# Autodesk Inventor assembly: STI Hybrid 98 Full Flange Assembly
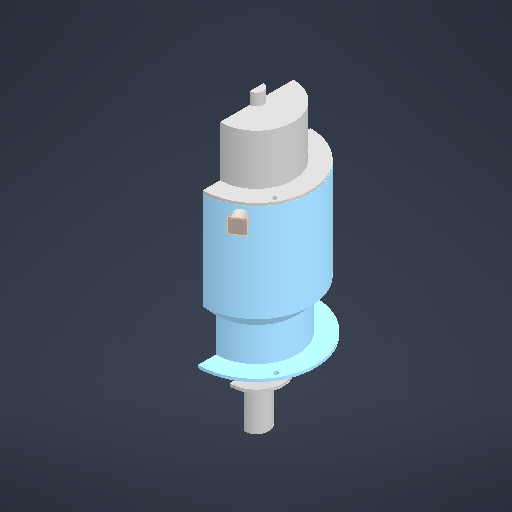
[picture p0: Inventor's stored thumbnail of the model, 512x512]
Saved by Autodesk Inventor 2026 (Build 300175050, 175E)
## iProperties
Created: 2025-07-03
Part Number: STI Hybrid 98 Full Flange Assembly
Document SubType Name: Assembly
Designer: user
Author: user
## Documents named in this file (3)
- C:\Projects\CryocoolerHybrid98\STI Hybrid 98 Full Flange Assembly.iam
- C:\Projects\CryocoolerHybrid98\STI Hybrid 98 Full Flange Cooling Shroud - Version 2.ipt
- C:\Projects\CryocoolerHybrid98\STI Hybrid 98 Cryocooler - Full Flange.ipt
## Components (2 placed, 2 different names)
1. STI Hybrid 98 Full Flange Cooling Shroud - Version 2:1 — Flush:1, Flush:2, Flush:3, Mate:1, Mate:2, Mate:3, Mate:4, Mate:5, Mate:6, Mate:7, Mate:8, Flush:4
2. STI Hybrid 98 Cryocooler - Full Flange:1 — Mate:5, Mate:6, Mate:7, Mate:8, Flush:4
## Relationships (12: Mate 8, Flush 4)
- Flush:1: STI Hybrid 98 Full Flange Cooling Shroud - Version 2:1
- Flush:2: STI Hybrid 98 Full Flange Cooling Shroud - Version 2:1
- Flush:3: STI Hybrid 98 Full Flange Cooling Shroud - Version 2:1
- Mate:1: STI Hybrid 98 Full Flange Cooling Shroud - Version 2:1
- Mate:2: STI Hybrid 98 Full Flange Cooling Shroud - Version 2:1
- Mate:3: STI Hybrid 98 Full Flange Cooling Shroud - Version 2:1
- Mate:4: STI Hybrid 98 Full Flange Cooling Shroud - Version 2:1
- Mate:5: STI Hybrid 98 Full Flange Cooling Shroud - Version 2:1 ↔ STI Hybrid 98 Cryocooler - Full Flange:1
- Mate:6: STI Hybrid 98 Full Flange Cooling Shroud - Version 2:1 ↔ STI Hybrid 98 Cryocooler - Full Flange:1
- Mate:7: STI Hybrid 98 Full Flange Cooling Shroud - Version 2:1 ↔ STI Hybrid 98 Cryocooler - Full Flange:1
- Mate:8: STI Hybrid 98 Full Flange Cooling Shroud - Version 2:1 ↔ STI Hybrid 98 Cryocooler - Full Flange:1
- Flush:4: STI Hybrid 98 Full Flange Cooling Shroud - Version 2:1 ↔ STI Hybrid 98 Cryocooler - Full Flange:1
